# Autodesk Inventor assembly: new_assembly
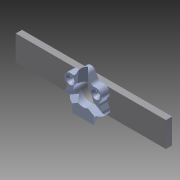
[picture p0: Inventor's stored thumbnail of the model, 180x180]
Saved by Autodesk Inventor 2011 (Build 150239000, 239)
## iProperties
Created: 2012-06-13
Part Number: new_assembly
Document SubType Name: Assembly
Designer: labuser
Author: labuser
## Documents named in this file (3)
- C:\Users\labuser\Documents\GitHub\kinematic_mount\magnet_chuck_redesign\new_assembly.iam
- C:\Users\labuser\Documents\GitHub\kinematic_mount\magnet_chuck_redesign\simple_chuck.ipt
- C:\Users\labuser\Documents\GitHub\kinematic_mount\magnet_chuck_redesign\TricornerSeat.ipt
## Components (2 placed, 2 different names)
1. simple_chuck:1 — Mate:1
2. TricornerSeat:1 — Mate:1
## Relationships (1: Mate 1)
- Mate:1: simple_chuck:1 ↔ TricornerSeat:1
